# Autodesk Inventor assembly: RAMPS Mount
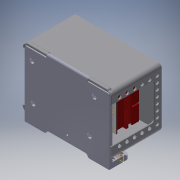
[picture p0: Inventor's stored thumbnail of the model, 180x180]
Saved by Autodesk Inventor 2018 (Build 220112000, 112)
## iProperties
Created: 2018-05-30
Part Number: RAMPS Mount
Document SubType Name: Assembly
Designer: Jasper
Author: Jasper
## Documents named in this file (5)
- D:\Jasper's Stuff\git_WSL\MEME_MACHINE\CAD\RAMPS Mount\RAMPS Mount.iam
- D:\Jasper's Stuff\git_WSL\MEME_MACHINE\CAD\RAMPS Mount\Mount.ipt
- D:\Jasper's Stuff\git_WSL\MEME_MACHINE\CAD\Vitamins\Arduino RAMPS combo.ipt
- D:\Jasper's Stuff\git_WSL\MEME_MACHINE\CAD\RAMPS Mount\Cover.ipt
- D:\Jasper's Stuff\git_WSL\MEME_MACHINE\CAD\Vitamins\RAMPS Smart Adapter.ipt
## Components (4 placed, 4 different names)
1. Mount:1 — Mate:1, Mate:2, Angle:1, Mate:5, Mate:6, Mate:7, Mate:8, Mate:9
2. Arduino RAMPS combo:1 — Mate:1, Mate:2, Angle:1, Flush:2, Mate:3, Mate:4
3. RAMPS Smart Adapter:1 — Flush:2, Mate:3, Mate:4
4. Cover:1 — Mate:5, Mate:6, Mate:7, Mate:8, Mate:9
## Relationships (11: Mate 9, Angle 1, Flush 1)
- Mate:1: Mount:1 ↔ Arduino RAMPS combo:1
- Mate:2: Mount:1 ↔ Arduino RAMPS combo:1
- Angle:1 (0 deg): Mount:1 ↔ Arduino RAMPS combo:1
- Flush:2: Arduino RAMPS combo:1 ↔ RAMPS Smart Adapter:1
- Mate:3: Arduino RAMPS combo:1 ↔ RAMPS Smart Adapter:1
- Mate:4: Arduino RAMPS combo:1 ↔ RAMPS Smart Adapter:1
- Mate:5: Mount:1 ↔ Cover:1
- Mate:6: Mount:1 ↔ Cover:1
- Mate:7: Mount:1 ↔ Cover:1
- Mate:8: Mount:1 ↔ Cover:1
- Mate:9: Mount:1 ↔ Cover:1
